# Autodesk Inventor assembly: ProbeAntenna_AdapterRWG_V1_Assembled
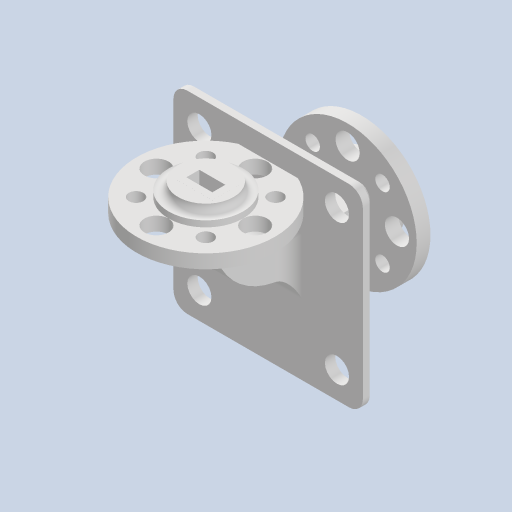
[picture p0: Inventor's stored thumbnail of the model, 512x512]
Saved by Autodesk Inventor 2023.2 (Build 272271000, 271)
## iProperties
Created: 2024-09-18
Part Number: ProbeAntenna_AdapterRWG_V1_Assembled
Document SubType Name: Assembly
Designer: Nils Bade
Author: Nils Bade
## Documents named in this file (3)
- C:\Users\nilsb\Documents\Inventor\Projektarbeit-Bade\RatRig_modified\ProbeHead\ProbeAntennas\ProbeAntenna_AdapterRWG_V1_Assembled.iam
- C:\Users\nilsb\Documents\Inventor\Projektarbeit-Bade\RatRig_modified\ProbeHead\ProbeAntennas\ProbeAntenna_AdapterRWG_V1.ipt
- C:\Users\nilsb\Documents\Inventor\Projektarbeit-Bade\RatRig_modified\ProbeHead\ProbeAntennas\IHFStandardParts\Hohlleiter-EndflanschV4.ipt
## Components (3 placed, 2 different names)
1. ProbeAntenna_AdapterRWG_V1:1 — Fluchtend:1, Fluchtend:2, Fluchtend:3, Fluchtend:4, Fluchtend:5, Passend:1
2. Hohlleiter-EndflanschV4:1 — Fluchtend:1, Fluchtend:2, Fluchtend:3
3. Hohlleiter-EndflanschV4:2 — Fluchtend:4, Fluchtend:5, Passend:1
## Relationships (6: Flush 5, Mate 1)
- Fluchtend:1 [Flush]: ProbeAntenna_AdapterRWG_V1:1 ↔ Hohlleiter-EndflanschV4:1
- Fluchtend:2 [Flush]: ProbeAntenna_AdapterRWG_V1:1 ↔ Hohlleiter-EndflanschV4:1
- Fluchtend:3 [Flush]: ProbeAntenna_AdapterRWG_V1:1 ↔ Hohlleiter-EndflanschV4:1
- Fluchtend:4 [Flush]: ProbeAntenna_AdapterRWG_V1:1 ↔ Hohlleiter-EndflanschV4:2
- Fluchtend:5 [Flush]: ProbeAntenna_AdapterRWG_V1:1 ↔ Hohlleiter-EndflanschV4:2
- Passend:1 [Mate]: ProbeAntenna_AdapterRWG_V1:1 ↔ Hohlleiter-EndflanschV4:2
